# Autodesk Inventor assembly: Stirlingmotor Bauguppe.0041
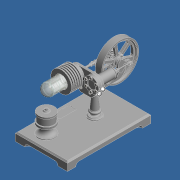
[picture p0: Inventor's stored thumbnail of the model, 180x180]
Saved by Autodesk Inventor 2018 (Build 220112000, 112)
## iProperties
Created: 2018-10-27
Material: Generisch
Document SubType Name: Assembly
Designer: M.Knabel
Description: Stirlingmotor
Author: M.Knabel
## Documents named in this file (39)
- C:\Inventor\StirlingKnabel\Daten\Stirlingmotor Bauguppe.iam
- C:\Inventor\StirlingKnabel\Daten\Grundplatte.ipt
- C:\Inventor\StirlingKnabel\Daten\Maschienensäule.ipt
- C:\Inventor\StirlingKnabel\Daten\Lagerarm.ipt
- C:\Inventor\StirlingKnabel\Daten\Zylinderplatte.ipt
- C:\Inventor\StirlingKnabel\Daten\Zylinder.ipt
- C:\Inventor\StirlingKnabel\Daten\Kühlkörper.ipt
- C:\Inventor\StirlingKnabel\Daten\Außenkolben.ipt
- C:\Inventor\StirlingKnabel\Daten\Rohr.ipt
- C:\Inventor\StirlingKnabel\Daten\Flansch.ipt
- C:\Inventor\StirlingKnabel\Daten\Schwungrad.ipt
- C:\Inventor\StirlingKnabel\Daten\Achse.ipt
- C:\Inventor\StirlingKnabel\Daten\Öler.ipt
- C:\Inventor\StirlingKnabel\Daten\Kurbel 19.ipt
- C:\Inventor\StirlingKnabel\Daten\Kurbel 20.ipt
- C:\Inventor\StirlingKnabel\Daten\Innenflansch.ipt
- C:\Inventor\StirlingKnabel\Daten\Verdrängerkolben.ipt
- C:\Inventor\StirlingKnabel\Daten\Kolbenstange.ipt
- C:\Inventor\StirlingKnabel\Daten\Lagerbuchse.ipt
- C:\Inventor\StirlingKnabel\Daten\Gabel.ipt
- C:\Inventor\StirlingKnabel\Daten\Pleuel.ipt
- C:\Inventor\StirlingKnabel\Daten\Pleuelkopf.ipt
- C:\Inventor\StirlingKnabel\Daten\Stangenkopf.ipt
- C:\Inventor\StirlingKnabel\Daten\Bolzen.ipt
- C:\Inventor\StirlingKnabel\Daten\Zapfen.ipt
- C:\Inventor\StirlingKnabel\Daten\Kolben.ipt
- C:\Inventor\StirlingKnabel\Daten\Brennerdeckel.ipt
- C:\Inventor\StirlingKnabel\Daten\Brennersockel.ipt
- C:\Inventor\StirlingKnabel\Daten\Brennertopf.ipt
- C:\Inventor\StirlingKnabel\Daten\Docht.ipt
- C:\Inventor\StirlingKnabel\Normteile\de-DE\ISO 1207(1)\DIN EN ISO 1207 - M3 x 10.ipt
- C:\Inventor\StirlingKnabel\Normteile\de-DE\DIN EN ISO 4017\DIN EN ISO 4017 - M3 x 12.ipt
- C:\Inventor\StirlingKnabel\Normteile\de-DE\DIN 913\DIN 913 - M3 x 3.ipt
- C:\Inventor\StirlingKnabel\Daten\Splint.ipt
- C:\Inventor\StirlingKnabel\Normteile\de-DE\ISO 1207(1)\DIN EN ISO 1207 - M4 x 25.ipt
- C:\Inventor\StirlingKnabel\Normteile\de-DE\DIN 913\DIN 913 - M3 x 6.ipt
- C:\Inventor\StirlingKnabel\Daten\Gummifüße.ipt
- C:\Inventor\StirlingKnabel\Daten\O-Ring.ipt
- C:\Inventor\StirlingKnabel\Daten\Gummi Schlauch.ipt
## Components (66 placed, 37 different names)
1. Grundplatte:1 — Passend:1, Passend:2, Winkel:1, Passend:71, Passend:72, Passend:73, Einfügen:8, Einfügen:9, Passend:107, Passend:108, Passend:109, Passend:110, Passend:111, Passend:112, Passend:113, Passend:114, Passend:115
2. Maschienensäule:1 — Passend:1, Passend:2, Winkel:1, Passend:3, Passend:4, Passend:5, Passend:6, Passend:7, Passend:8, Passend:80
3. Lagerarm:1 — Passend:3, Passend:4, Passend:5, Passend:11, Passend:28, Passend:31, Passend:32, Passend:35, Passend:81, Passend:82, Passend:83, Passend:106
4. Lagerarm:2 — Passend:6, Passend:7, Passend:8, Passend:9, Passend:10, Passend:29, Passend:30, Passend:33, Passend:34, Passend:37, Animation, Passend:84, Passend:85, Passend:86, Passend:87
5. Zylinderplatte:1 — Passend:9, Passend:10, Passend:11, Passend:12, Passend:13, Passend:14, Passend:15, Passend:16, Passend:17, Einfügen:2, Passend:49, Passend:51, Passend:88, Passend:89, Passend:90, Passend:91, Passend:96, Passend:97
6. Zylinder:1 — Passend:12, Passend:13, Passend:52
7. Kühlkörper:1 — Passend:14, Passend:15, Passend:16, Passend:17, Passend:18, Passend:19, Passend:20, Passend:21, Passend:41, Passend:121
8. Außenkolben:1 — Passend:18, Passend:19
9. Rohr:1 — Passend:20, Passend:21, Passend:50, Passend:120
10. Flansch:1 — Passend:25, Passend:26, Passend:49, Passend:51, Passend:94, Passend:95
11. Rohr:2 — Passend:25, Passend:26, Passend:50
12. Schwungrad:1 — Passend:28, Winkel:4, Passend:100, Passend:101, Passend:106
13. Achse:1 — Passend:29, Passend:30, Passend:36, Passend:38
14. Öler:1 — Passend:31, Passend:32
15. Öler:2 — Passend:33, Passend:34
16. Kurbel:1 — Passend:35, Passend:36, Passend:57, Passend:118, Winkel:8, Passend:124
17. Kurbel:2 — Passend:37, Passend:38, Passend:60, Winkel:4, Animation, Passend:119, Winkel:8
18. Innenflansch:1 — Passend:39, Passend:40, Einfügen:1, Passend:122, Passend:123, Tangential:1, Tangential:2
19. Duranglas:1 — Passend:39, Passend:40, Passend:41
20. Kolbenstange:1 — Einfügen:1, Einfügen:3
21. Lagerbuchse:1 — Einfügen:2
22. Gabel:1 — Einfügen:3, Passend:45, Passend:46, Passend:63, Winkel:7
23. Bolzen:1 — Passend:45, Passend:46, Passend:61, Passend:102, Passend:103
24. Kolben:1 — Passend:52, Passend:55, Passend:56, Passend:68
25. Pleuel:2 — Fluchtend:1, Passend:54
26. Pleuelkopf:2 — Passend:57, Passend:58, Passend:59
27. Zapfen:2 — Passend:58, Passend:59
28. Gabel:2 — Fluchtend:1, Passend:54, Passend:55, Passend:56, Passend:67, Winkel:6
29. Pleuel:3 — Passend:64, Passend:65, Passend:66
30. Pleuelkopf:3 — Passend:60, Passend:62, Passend:65, Passend:69, Passend:70
31. Stangenkopf:1 — Passend:61, Passend:62, Passend:63, Passend:64, Passend:66
32. Bolzen:2 — Passend:67, Passend:68, Passend:104, Passend:105
33. Zapfen:3 — Passend:69, Passend:70
34. Brennerdeckel:1 — Passend:76, Passend:77, Passend:78, Passend:107
35. Brennersockel:1 — Passend:71, Passend:72, Passend:73, Passend:74, Passend:75
36. Brennertopf:1 — Passend:74, Passend:75, Passend:76, Passend:77, Passend:79
37. Docht:1 — Passend:78, Passend:79
38. DIN EN ISO 1207 M3 x 10:1 — Passend:80, Passend:81
39. DIN EN ISO 1207 M3 x 10:2 — Passend:82, Passend:83
40. DIN EN ISO 1207 M3 x 10:3 — Passend:84, Passend:85
41. DIN EN ISO 1207 M3 x 10:4 — Passend:86, Passend:87
42. DIN EN ISO 1207 M4 x 25:2 — Einfügen:8
43. DIN EN ISO 1207 M4 x 25:1 — Einfügen:9
44. DIN EN ISO 1207 M3 x 10:5 — Passend:88, Passend:89
45. DIN EN ISO 1207 M3 x 10:6 — Passend:90, Passend:91
46. DIN 913 M3 x 6:1 — Passend:100, Passend:101
47. Splint:1 — Passend:102, Passend:103, Winkel:7
48. Splint:2 — Passend:104, Passend:105, Winkel:6
49. Gummifüße:1 — Passend:114, Passend:115
50. Gummifüße:2 — Passend:112, Passend:113
51. Gummifüße:3 — Passend:110, Passend:111
52. Gummifüße:4 — Passend:108, Passend:109
53. O-Ring:1 — Passend:123, Tangential:2
54. O-Ring:2 — Passend:122, Tangential:1
55. DIN 913 M3 x 3:3 — Passend:118, Passend:124
56. DIN 913 M3 x 3:4 — Passend:119
57. Gummi Schlauch:1 — Passend:120, Passend:121
58. DIN EN ISO 4017 M3 x 12:2 — Passend:94, Passend:95
59. DIN EN ISO 4017 M3 x 12:3
60. DIN EN ISO 4017 M3 x 12:4
61. DIN EN ISO 4017 M3 x 12:5
62. DIN EN ISO 4017 M3 x 12:6
63. DIN EN ISO 4017 M3 x 12:7
64. DIN EN ISO 4017 M3 x 12:8 — Passend:96, Passend:97
65. DIN EN ISO 4017 M3 x 12:9
66. DIN EN ISO 4017 M3 x 12:10
## Component patterns: (6 elements, first: DIN EN ISO 4017 M3 x 12:2), (3 elements, first: DIN EN ISO 4017 M3 x 12:8)
## Relationships (123: Mate 108, Angle 6, Insert 6, Tangent 2, Flush 1)
- Passend:1 [Mate]: Grundplatte:1 ↔ Maschienensäule:1
- Passend:2 [Mate]: Grundplatte:1 ↔ Maschienensäule:1
- Winkel:1 [Angle] (0 deg): Grundplatte:1 ↔ Maschienensäule:1
- Passend:3 [Mate]: Maschienensäule:1 ↔ Lagerarm:1
- Passend:4 [Mate]: Maschienensäule:1 ↔ Lagerarm:1
- Passend:5 [Mate]: Maschienensäule:1 ↔ Lagerarm:1
- Passend:6 [Mate]: Maschienensäule:1 ↔ Lagerarm:2
- Passend:7 [Mate]: Maschienensäule:1 ↔ Lagerarm:2
- Passend:8 [Mate]: Maschienensäule:1 ↔ Lagerarm:2
- Passend:9 [Mate]: Lagerarm:2 ↔ Zylinderplatte:1
- Passend:10 [Mate]: Lagerarm:2 ↔ Zylinderplatte:1
- Passend:11 [Mate]: Lagerarm:1 ↔ Zylinderplatte:1
- Passend:12 [Mate]: Zylinderplatte:1 ↔ Zylinder:1
- Passend:13 [Mate]: Zylinderplatte:1 ↔ Zylinder:1
- Passend:14 [Mate]: Zylinderplatte:1 ↔ Kühlkörper:1
- Passend:15 [Mate]: Zylinderplatte:1 ↔ Kühlkörper:1
- Passend:16 [Mate]: Zylinderplatte:1 ↔ Kühlkörper:1
- Passend:17 [Mate]: Zylinderplatte:1 ↔ Kühlkörper:1
- Passend:18 [Mate]: Kühlkörper:1 ↔ Außenkolben:1
- Passend:19 [Mate]: Kühlkörper:1 ↔ Außenkolben:1
- Passend:20 [Mate]: Kühlkörper:1 ↔ Rohr:1
- Passend:21 [Mate]: Kühlkörper:1 ↔ Rohr:1
- Passend:25 [Mate]: Flansch:1 ↔ Rohr:2
- Passend:26 [Mate]: Flansch:1 ↔ Rohr:2
- Passend:28 [Mate]: Lagerarm:1 ↔ Schwungrad:1
- Passend:29 [Mate] (-32 mm): Lagerarm:2 ↔ Achse:1
- Passend:30 [Mate]: Lagerarm:2 ↔ Achse:1
- Passend:31 [Mate]: Lagerarm:1 ↔ Öler:1
- Passend:32 [Mate]: Lagerarm:1 ↔ Öler:1
- Passend:33 [Mate]: Lagerarm:2 ↔ Öler:2
- Passend:34 [Mate]: Lagerarm:2 ↔ Öler:2
- Passend:35 [Mate]: Lagerarm:1 ↔ Kurbel:1
- Passend:36 [Mate]: Achse:1 ↔ Kurbel:1
- Passend:37 [Mate]: Lagerarm:2 ↔ Kurbel:2
- Passend:38 [Mate]: Achse:1 ↔ Kurbel:2
- Passend:39 [Mate]: Innenflansch:1 ↔ Duranglas:1
- Passend:40 [Mate]: Innenflansch:1 ↔ Duranglas:1
- Einfügen:1 [Insert]: Innenflansch:1 ↔ Kolbenstange:1
- Einfügen:2 [Insert]: Zylinderplatte:1 ↔ Lagerbuchse:1
- Passend:41 [Mate]: Kühlkörper:1 ↔ Duranglas:1
- Einfügen:3 [Insert]: Kolbenstange:1 ↔ Gabel:1
- Passend:45 [Mate]: Gabel:1 ↔ Bolzen:1
- Passend:46 [Mate]: Gabel:1 ↔ Bolzen:1
- Passend:49 [Mate]: Zylinderplatte:1 ↔ Flansch:1
- Passend:50 [Mate]: Rohr:1 ↔ Rohr:2
- Passend:51 [Mate]: Zylinderplatte:1 ↔ Flansch:1
- Passend:52 [Mate]: Zylinder:1 ↔ Kolben:1
- [Insert]: Pleuel:2 ↔ Pleuelkopf:2
- Fluchtend:1 [Flush]: Pleuel:2 ↔ Gabel:2
- Passend:54 [Mate]: Pleuel:2 ↔ Gabel:2
- Passend:55 [Mate]: Kolben:1 ↔ Gabel:2
- Passend:56 [Mate]: Kolben:1 ↔ Gabel:2
- Passend:57 [Mate]: Kurbel:1 ↔ Pleuelkopf:2
- Passend:58 [Mate]: Pleuelkopf:2 ↔ Zapfen:2
- Passend:59 [Mate]: Pleuelkopf:2 ↔ Zapfen:2
- Passend:60 [Mate]: Kurbel:2 ↔ Pleuelkopf:3
- Passend:61 [Mate]: Bolzen:1 ↔ Stangenkopf:1
- Passend:62 [Mate]: Pleuelkopf:3 ↔ Stangenkopf:1
- Passend:63 [Mate]: Gabel:1 ↔ Stangenkopf:1
- Passend:64 [Mate]: Pleuel:3 ↔ Stangenkopf:1
- Passend:65 [Mate] (-3 mm): Pleuel:3 ↔ Pleuelkopf:3
- Passend:66 [Mate] (-3 mm): Pleuel:3 ↔ Stangenkopf:1
- Passend:67 [Mate]: Gabel:2 ↔ Bolzen:2
- Passend:68 [Mate]: Kolben:1 ↔ Bolzen:2
- Passend:69 [Mate]: Pleuelkopf:3 ↔ Zapfen:3
- Passend:70 [Mate]: Pleuelkopf:3 ↔ Zapfen:3
- Passend:71 [Mate]: Grundplatte:1 ↔ Brennersockel:1
- Passend:72 [Mate]: Grundplatte:1 ↔ Brennersockel:1
- Passend:73 [Mate]: Grundplatte:1 ↔ Brennersockel:1
- Passend:74 [Mate]: Brennersockel:1 ↔ Brennertopf:1
- Passend:75 [Mate]: Brennersockel:1 ↔ Brennertopf:1
- Passend:76 [Mate]: Brennerdeckel:1 ↔ Brennertopf:1
- Passend:77 [Mate]: Brennerdeckel:1 ↔ Brennertopf:1
- Winkel:4 [Angle] (310 deg): Schwungrad:1 ↔ Kurbel:2
- Animation [Angle] (270 deg): Lagerarm:2 ↔ Kurbel:2
- Passend:78 [Mate]: Brennerdeckel:1 ↔ Docht:1
- Passend:79 [Mate]: Brennertopf:1 ↔ Docht:1
- Passend:80 [Mate]: Maschienensäule:1 ↔ DIN EN ISO 1207 M3 x 10:1
- Passend:81 [Mate]: Lagerarm:1 ↔ DIN EN ISO 1207 M3 x 10:1
- Passend:82 [Mate]: Lagerarm:1 ↔ DIN EN ISO 1207 M3 x 10:2
- Passend:83 [Mate]: Lagerarm:1 ↔ DIN EN ISO 1207 M3 x 10:2
- Passend:84 [Mate]: Lagerarm:2 ↔ DIN EN ISO 1207 M3 x 10:3
- Passend:85 [Mate]: Lagerarm:2 ↔ DIN EN ISO 1207 M3 x 10:3
- Passend:86 [Mate]: Lagerarm:2 ↔ DIN EN ISO 1207 M3 x 10:4
- Passend:87 [Mate]: Lagerarm:2 ↔ DIN EN ISO 1207 M3 x 10:4
- Einfügen:8 [Insert]: Grundplatte:1 ↔ DIN EN ISO 1207 M4 x 25:2
- Einfügen:9 [Insert]: Grundplatte:1 ↔ DIN EN ISO 1207 M4 x 25:1
- Passend:88 [Mate]: Zylinderplatte:1 ↔ DIN EN ISO 1207 M3 x 10:5
- Passend:89 [Mate]: Zylinderplatte:1 ↔ DIN EN ISO 1207 M3 x 10:5
- Passend:90 [Mate]: Zylinderplatte:1 ↔ DIN EN ISO 1207 M3 x 10:6
- Passend:91 [Mate]: Zylinderplatte:1 ↔ DIN EN ISO 1207 M3 x 10:6
- Passend:94 [Mate]: Flansch:1 ↔ DIN EN ISO 4017 M3 x 12:2
- Passend:95 [Mate]: Flansch:1 ↔ DIN EN ISO 4017 M3 x 12:2
- Passend:96 [Mate]: Zylinderplatte:1 ↔ DIN EN ISO 4017 M3 x 12:8
- Passend:97 [Mate]: Zylinderplatte:1 ↔ DIN EN ISO 4017 M3 x 12:8
- Passend:100 [Mate]: Schwungrad:1 ↔ DIN 913 M3 x 6:1
- Passend:101 [Mate] (8 mm): Schwungrad:1 ↔ DIN 913 M3 x 6:1
- Passend:102 [Mate]: Bolzen:1 ↔ Splint:1
- Passend:103 [Mate] (2.5 mm): Bolzen:1 ↔ Splint:1
- Passend:104 [Mate]: Bolzen:2 ↔ Splint:2
- Passend:105 [Mate] (2.5 mm): Bolzen:2 ↔ Splint:2
- Winkel:6 [Angle] (0 deg): Gabel:2 ↔ Splint:2
- Winkel:7 [Angle] (180 deg): Gabel:1 ↔ Splint:1
- Passend:106 [Mate] (0.5 mm): Lagerarm:1 ↔ Schwungrad:1
- Passend:107 [Mate] (-33.5 mm): Grundplatte:1 ↔ Brennerdeckel:1
- Passend:108 [Mate]: Grundplatte:1 ↔ Gummifüße:4
- Passend:109 [Mate]: Grundplatte:1 ↔ Gummifüße:4
- Passend:110 [Mate]: Grundplatte:1 ↔ Gummifüße:3
- Passend:111 [Mate]: Grundplatte:1 ↔ Gummifüße:3
- Passend:112 [Mate]: Grundplatte:1 ↔ Gummifüße:2
- Passend:113 [Mate]: Grundplatte:1 ↔ Gummifüße:2
- Passend:114 [Mate]: Grundplatte:1 ↔ Gummifüße:1
- Passend:115 [Mate]: Grundplatte:1 ↔ Gummifüße:1
- Passend:118 [Mate]: Kurbel:1 ↔ DIN 913 M3 x 3:3
- Passend:119 [Mate]: Kurbel:2 ↔ DIN 913 M3 x 3:4
- Passend:120 [Mate]: Rohr:1 ↔ Gummi Schlauch:1
- Passend:121 [Mate] (19.5 mm): Kühlkörper:1 ↔ Gummi Schlauch:1
- Passend:122 [Mate]: Innenflansch:1 ↔ O-Ring:2
- Passend:123 [Mate]: Innenflansch:1 ↔ O-Ring:1
- Tangential:1: Innenflansch:1 ↔ O-Ring:2
- Tangential:2: Innenflansch:1 ↔ O-Ring:1
- Winkel:8 [Angle] (90 deg): Kurbel:1 ↔ Kurbel:2
- Passend:124 [Mate]: Kurbel:1 ↔ DIN 913 M3 x 3:3
## Named parameters: d70_d55 = 0 mm
